# Autodesk Inventor assembly: front_assembly
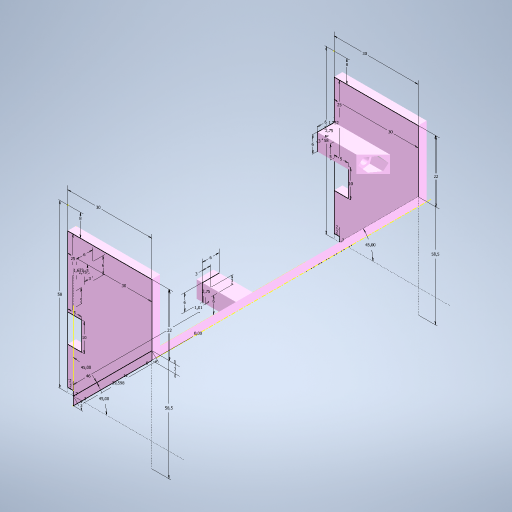
[picture p0: Inventor's stored thumbnail of the model, 512x512]
Saved by Autodesk Inventor 2023 (Build 270158000, 158)
## iProperties
Created: 2023-03-01
Part Number: front_assembly
Document SubType Name: Assembly
Designer: Eryk
Author: Eryk
## Documents named in this file (4)
- C:\Users\Eryk\Documents\PEM\front_assembly.iam
- C:\Users\Eryk\Documents\PEM\front.ipt
- C:\Users\Eryk\Documents\PEM\side_wall.ipt
- C:\Users\Eryk\Documents\PEM\side_wall_left.ipt
## Components (3 placed, 3 different names)
1. front:1 — Mate:4, Mate:5, Mate:6, Mate:7, Mate:8, Mate:9
2. side_wall:2 — Mate:4, Mate:5, Mate:6
3. side_wall_left:1 — Mate:7, Mate:8, Mate:9
## Relationships (6: Mate 6)
- Mate:4: front:1 ↔ side_wall:2
- Mate:5: front:1 ↔ side_wall:2
- Mate:6: front:1 ↔ side_wall:2
- Mate:7: front:1 ↔ side_wall_left:1
- Mate:8: front:1 ↔ side_wall_left:1
- Mate:9: front:1 ↔ side_wall_left:1
